# Autodesk Inventor assembly: Nanoscopy-on-a-cheap_v3_mono
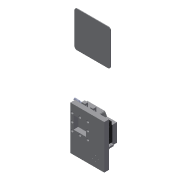
[picture p0: Inventor's stored thumbnail of the model, 180x180]
Saved by Autodesk Inventor 2019 (Build 230136000, 136)
## iProperties
Created: 2019-05-02
Part Number: Nanoscopy-on-a-cheap_v3_mono
Document SubType Name: Assembly
Designer: diederichbenedict
Author: diederichbenedict
## Documents named in this file (12)
- C:\Users\diederichbenedict\Dropbox\Dokumente\Promotion\PROJECTS\STORMoChip\INVENTOR\Nanoscopy-on-a-cheap\Nanoscopy-on-a-cheap_v3_mono.iam
- C:\Users\diederichbenedict\Dropbox\Dokumente\Promotion\PROJECTS\STORMoChip\INVENTOR\Nanoscopy-on-a-cheap\00_ZEISS_Axiotech_Plate.ipt
- C:\Users\diederichbenedict\Dropbox\Dokumente\Promotion\PROJECTS\STORMoChip\INVENTOR\Nanoscopy-on-a-cheap\00_XY_stage-CHUO_SEIKI_LD-647-R1.iam
- C:\Users\diederichbenedict\Dropbox\Dokumente\Promotion\PROJECTS\STORMoChip\INVENTOR\Nanoscopy-on-a-cheap\Assembly_Lasergroup_wPickup_v1.iam
- C:\Users\diederichbenedict\Dropbox\Dokumente\Promotion\PROJECTS\STORMoChip\INVENTOR\Nanoscopy-on-a-cheap\00_Microscope_Objective.ipt
- C:\Users\diederichbenedict\Dropbox\Dokumente\Promotion\PROJECTS\STORMoChip\INVENTOR\Nanoscopy-on-a-cheap\10_Adapter_Laser_XY_left.ipt
- C:\Users\diederichbenedict\Dropbox\Dokumente\Promotion\PROJECTS\STORMoChip\INVENTOR\Nanoscopy-on-a-cheap\02_Nanoscopy_Chip.ipt
- C:\Users\diederichbenedict\Dropbox\Dokumente\Promotion\PROJECTS\STORMoChip\INVENTOR\Nanoscopy-on-a-cheap\10_Baseplate.ipt
- C:\Users\diederichbenedict\Dropbox\Dokumente\Promotion\PROJECTS\STORMoChip\INVENTOR\Nanoscopy-on-a-cheap\00_Baseplate_Axiotech.ipt
- C:\Users\diederichbenedict\Dropbox\Dokumente\Promotion\PROJECTS\STORMoChip\INVENTOR\Nanoscopy-on-a-cheap\10_Baseplate_Axiotech_mono.ipt
- C:\Users\diederichbenedict\Dropbox\Dokumente\Promotion\PROJECTS\STORMoChip\INVENTOR\Nanoscopy-on-a-cheap\00_Metalsheet_1mm_30x40.ipt
- C:\Users\diederichbenedict\Dropbox\Dokumente\Promotion\PROJECTS\STORMoChip\INVENTOR\Nanoscopy-on-a-cheap\102_Z_Focus_CCTV_Camera.ipt
## Components (11 placed, 11 different names)
1. 00_ZEISS_Axiotech_Plate:1 — Mate:13
2. 00_XY_stage-CHUO_SEIKI_LD-647-R1:1 [sub-assembly] — Flush:6, Flush:11, Flush:12, Flush:22, Flush:23, Flush:24, Flush:25, Flush:26
3. Assembly_Lasergroup_wPickup_v1:2 [sub-assembly] — Flush:6, Mate:7, Mate:8
4. 02_Nanoscopy_Chip:1 — Mate:17
5. 00_Microscope_Objective:1 — Mate:7, Mate:8, Mate:13
6. 10_Adapter_Laser_XY_left:1 — Flush:11, Flush:12
7. 10_Baseplate:1 — Flush:22, Flush:23
8. 00_Baseplate_Axiotech:1
9. 10_Baseplate_Axiotech_mono:1 — Flush:24, Flush:25, Flush:26, Angle:3, Flush:27, Flush:28, Flush:29
10. 00_Metalsheet_1mm_30x40:1 — Angle:3, Mate:17
11. 102_Z_Focus_CCTV_Camera:1 — Flush:27, Flush:28, Flush:29
## Relationships (18: Flush 11, Mate 4, Angle 2, Insert 1)
- Flush:6: 00_XY_stage-CHUO_SEIKI_LD-647-R1:1 ↔ Assembly_Lasergroup_wPickup_v1:2
- Mate:7 (30 mm): Assembly_Lasergroup_wPickup_v1:2 ↔ 00_Microscope_Objective:1
- Mate:8 (-16 mm): Assembly_Lasergroup_wPickup_v1:2 ↔ 00_Microscope_Objective:1
- Flush:11: 00_XY_stage-CHUO_SEIKI_LD-647-R1:1 ↔ 10_Adapter_Laser_XY_left:1
- Flush:12: 00_XY_stage-CHUO_SEIKI_LD-647-R1:1 ↔ 10_Adapter_Laser_XY_left:1
- Mate:13 (30 mm): 00_ZEISS_Axiotech_Plate:1 ↔ 00_Microscope_Objective:1
- [Insert] (5 mm): 02_Nanoscopy_Chip:1 ↔ 00_Microscope_Objective:1
- [Angle] (180 deg): 02_Nanoscopy_Chip:1 ↔ 10_Adapter_Laser_XY_left:1
- Flush:22: 00_XY_stage-CHUO_SEIKI_LD-647-R1:1 ↔ 10_Baseplate:1
- Flush:23: 00_XY_stage-CHUO_SEIKI_LD-647-R1:1 ↔ 10_Baseplate:1
- Flush:24: 00_XY_stage-CHUO_SEIKI_LD-647-R1:1 ↔ 10_Baseplate_Axiotech_mono:1
- Flush:25: 00_XY_stage-CHUO_SEIKI_LD-647-R1:1 ↔ 10_Baseplate_Axiotech_mono:1
- Flush:26: 00_XY_stage-CHUO_SEIKI_LD-647-R1:1 ↔ 10_Baseplate_Axiotech_mono:1
- Angle:3 (180 deg): 10_Baseplate_Axiotech_mono:1 ↔ 00_Metalsheet_1mm_30x40:1
- Mate:17: 02_Nanoscopy_Chip:1 ↔ 00_Metalsheet_1mm_30x40:1
- Flush:27 (3 mm): 10_Baseplate_Axiotech_mono:1 ↔ 102_Z_Focus_CCTV_Camera:1
- Flush:28 (10 mm): 10_Baseplate_Axiotech_mono:1 ↔ 102_Z_Focus_CCTV_Camera:1
- Flush:29 (10 mm): 10_Baseplate_Axiotech_mono:1 ↔ 102_Z_Focus_CCTV_Camera:1
